# Autodesk Inventor assembly: MountA
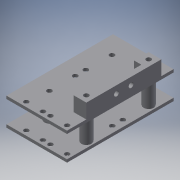
[picture p0: Inventor's stored thumbnail of the model, 180x180]
Saved by Autodesk Inventor 2018 (Build 220112000, 112)
## iProperties
Created: 2018-05-09
Part Number: MountA
Document SubType Name: Assembly
Designer: s4321966
Author: s4321966
## Documents named in this file (4)
- H:\Inventor-Workspace\METR4901\PCB Mount\MountA.iam
- H:\Inventor-Workspace\METR4901\PCB Mount\mountBrace.ipt
- H:\Inventor-Workspace\METR4901\PCB Mount\mountMount.ipt
- H:\Inventor-Workspace\METR4901\PCB Mount\mountPCB.ipt
## Components (3 placed, 3 different names)
1. mountBrace:1 — Mate:1, Tangent:1, Tangent:2
2. mountMount:1 — Mate:1, Tangent:1, Tangent:2, Mate:2, Flush:1, Flush:2
3. mountPCB:1 — Mate:2, Flush:1, Flush:2
## Relationships (6: Mate 2, Tangent 2, Flush 2)
- Mate:1: mountBrace:1 ↔ mountMount:1
- Tangent:1: mountBrace:1 ↔ mountMount:1
- Tangent:2: mountBrace:1 ↔ mountMount:1
- Mate:2: mountMount:1 ↔ mountPCB:1
- Flush:1: mountMount:1 ↔ mountPCB:1
- Flush:2: mountMount:1 ↔ mountPCB:1
